# Autodesk Inventor assembly: 39079
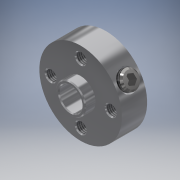
[picture p0: Inventor's stored thumbnail of the model, 180x180]
Saved by Autodesk Inventor 2017.1 (Build 211199000, 199)
## iProperties
Category: Wheel Hardware
Company: Autodesk Inc.
Created: 2017-01-02
Part Number: 39079
Document SubType Name: Assembly
Designer: Autodesk Inc.
Catalog Web Link: http://www.tetrixrobotics.com/TETRIX_Motor_Shaft_Hubs
Vendor: Tetrix
Author: Autodesk Inc.
## Documents named in this file (3)
- D:\FIRST\FTC KOP 2017\FTC 2017 KOP\Tetrix\Tetrix_39079.iam
- D:\FIRST\FTC KOP 2017\FTC 2017 KOP\Tetrix\Tetrix_739079_Collar.ipt
- D:\FIRST\FTC KOP 2017\FTC 2017 KOP\Tetrix\Tetrix_739079_Screw.ipt
## Components (2 placed, 2 different names)
1. Tetrix_39079_Collar:1 — Mate:1
2. Tetrix_39079_Screw:1 — Mate:1
## Relationships (1: Mate 1)
- Mate:1: Tetrix_39079_Collar:1 ↔ Tetrix_39079_Screw:1
